# Autodesk Inventor assembly: Hektor3D
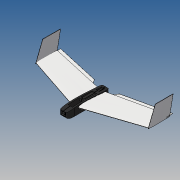
[picture p0: Inventor's stored thumbnail of the model, 180x180]
Saved by Autodesk Inventor 2019.4 (Build 234330000, 330)
## iProperties
Part Number: Hektor3D
Document SubType Name: Assembly
Designer: Admin
Mass: 25466.1 g
Surface Area: 19314.4 cm^2
Volume: 16701.2 cm^3
Density: 1.52481 g/cm^3
Revision: -
VAULT_Status: in Bearbeitung
Gewicht: 25,466 kg
InventorVersion: 2019.4
Author: Admin
## Documents named in this file (8)
- C:\Users\tonn\Documents\GitHub\CAD_Elements\CAD\Hektor\Hektor_3D\Hektor3D.iam
- HEKTOR3D_HEKTOR3D.IAM
- C:\Users\tonn\Documents\GitHub\CAD_Elements\CAD\Hektor\Hektor_3D\Rumpfhälfte.ipt
- C:\Users\tonn\Documents\GitHub\CAD_Elements\CAD\Hektor\Hektor_3D\Rumpfhälfte1.ipt
- C:\Users\tonn\Documents\GitHub\CAD_Elements\CAD\Hektor\Hektor_3D\wing_r.ipt
- C:\Users\tonn\Documents\GitHub\CAD_Elements\CAD\Hektor\Hektor_3D\Wing_L.ipt
- C:\Users\tonn\Documents\GitHub\CAD_Elements\CAD\Hektor\Hektor_3D\Winlet_R.ipt
- C:\Users\tonn\Documents\GitHub\CAD_Elements\CAD\Hektor\Hektor_3D\Winglet_L.ipt
## Components (6 placed, 6 different names)
1. RUMPFHÄLFTE_RUMPFHÄLFTE:1 — Fluchtend:1, Fluchtend:2, Fluchtend:3, Passend:3, Passend:4, Passend:7
2. RUMPFHÄLFTE1_RUMPFHÄLFTE1:1 — Passend:1, Fluchtend:4, Passend:2, Passend:5, Passend:6, Passend:8
3. WING_R_WING_R:1 — Passend:3, Passend:4, Passend:7, Passend:9, Fluchtend:11, Fluchtend:12
4. WING_L_WING_L:1 — Passend:5, Passend:6, Passend:8
5. WINLET_R_WINLET_R:1 — Passend:9, Fluchtend:11, Fluchtend:12
6. WINGLET_L_WINGLET_L:1
## Relationships (15: Mate 9, Flush 6)
- Fluchtend:1 [Flush] (2.5 mm): RUMPFHÄLFTE_RUMPFHÄLFTE:1
- Fluchtend:2 [Flush]: RUMPFHÄLFTE_RUMPFHÄLFTE:1
- Fluchtend:3 [Flush] (75 mm): RUMPFHÄLFTE_RUMPFHÄLFTE:1
- Passend:1 [Mate] (-75 mm): RUMPFHÄLFTE1_RUMPFHÄLFTE1:1
- Fluchtend:4 [Flush]: RUMPFHÄLFTE1_RUMPFHÄLFTE1:1
- Passend:2 [Mate] (2.5 mm): RUMPFHÄLFTE1_RUMPFHÄLFTE1:1
- Passend:3 [Mate]: RUMPFHÄLFTE_RUMPFHÄLFTE:1 ↔ WING_R_WING_R:1
- Passend:4 [Mate]: RUMPFHÄLFTE_RUMPFHÄLFTE:1 ↔ WING_R_WING_R:1
- Passend:5 [Mate]: RUMPFHÄLFTE1_RUMPFHÄLFTE1:1 ↔ WING_L_WING_L:1
- Passend:6 [Mate]: RUMPFHÄLFTE1_RUMPFHÄLFTE1:1 ↔ WING_L_WING_L:1
- Passend:7 [Mate]: RUMPFHÄLFTE_RUMPFHÄLFTE:1 ↔ WING_R_WING_R:1
- Passend:8 [Mate]: RUMPFHÄLFTE1_RUMPFHÄLFTE1:1 ↔ WING_L_WING_L:1
- Passend:9 [Mate] (-8 mm): WING_R_WING_R:1 ↔ WINLET_R_WINLET_R:1
- Fluchtend:11 [Flush] (-750 mm): WING_R_WING_R:1 ↔ WINLET_R_WINLET_R:1
- Fluchtend:12 [Flush] (205 mm): WING_R_WING_R:1 ↔ WINLET_R_WINLET_R:1
## Named parameters: Gewicht = 25.4661
note: some values were not read from the file. Shown as the stored number, unit unknown: "Gewicht".
